# Autodesk Inventor assembly: Motherboard_assembly
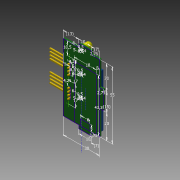
[picture p0: Inventor's stored thumbnail of the model, 180x180]
Saved by Autodesk Inventor 2016 (Build 200138000, 138)
## iProperties
Created: 2015-06-12
Part Number: Motherboard_assembly
Document SubType Name: Assembly
Designer: Openlab
Author: Openlab
## Documents named in this file (4)
- D:\Alexey\HS-Spectrophotometer\parts\Paris\Microcontroller_board_assumbly.iam
- D:\Alexey\HS-Spectrophotometer\parts\Paris\Microcontroller_board.ipt
- D:\Alexey\HS-Spectrophotometer\parts\Common\Pin-connector-angled-4.iam
- D:\Alexey\HS-Spectrophotometer\parts\Common\LED.ipt
## Components (6 placed, 3 different names)
1. Microcontroller_board:1 — Mate:1, Mate:4, Mate:5, Mate:6, Mate:7, Mate:8, Mate:9, Mate:11, Mate:12, Mate:13, Mate:14, Mate:15
2. Pin-connector-angled-4:1 [sub-assembly] — Mate:1, Mate:7, Mate:8
3. Pin-connector-angled-4:2 [sub-assembly] — Mate:4, Mate:5, Mate:6
4. LED:1 — Mate:9, Mate:15
5. LED:2 — Mate:13, Mate:14
6. LED:3 — Mate:11, Mate:12
## Relationships (12: Mate 12)
- Mate:1: Microcontroller_board:1 ↔ Pin-connector-angled-4:1
- Mate:4: Microcontroller_board:1 ↔ Pin-connector-angled-4:2
- Mate:5: Microcontroller_board:1 ↔ Pin-connector-angled-4:2
- Mate:6: Microcontroller_board:1 ↔ Pin-connector-angled-4:2
- Mate:7: Microcontroller_board:1 ↔ Pin-connector-angled-4:1
- Mate:8: Microcontroller_board:1 ↔ Pin-connector-angled-4:1
- Mate:9: Microcontroller_board:1 ↔ LED:1
- Mate:11: Microcontroller_board:1 ↔ LED:3
- Mate:12 (8 mm): Microcontroller_board:1 ↔ LED:3
- Mate:13: Microcontroller_board:1 ↔ LED:2
- Mate:14 (8 mm): Microcontroller_board:1 ↔ LED:2
- Mate:15 (8 mm): Microcontroller_board:1 ↔ LED:1
